# Autodesk Inventor assembly: GX 100
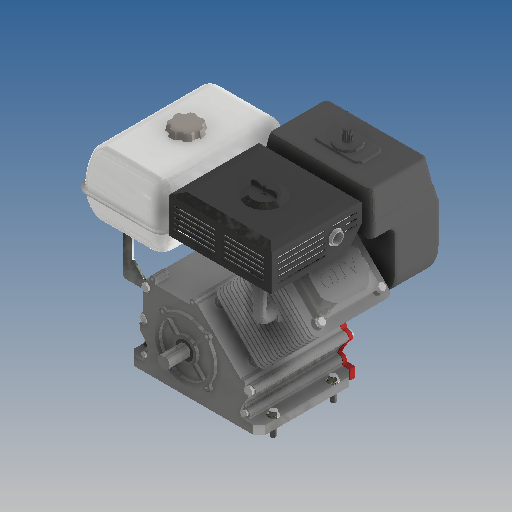
[picture p0: Inventor's stored thumbnail of the model, 512x512]
Saved by Autodesk Inventor 2021.1 (Build 251245000, 245)
## iProperties
Created: 2020-09-03
Part Number: GX 100
Document SubType Name: Assembly
Designer: alid
Description: Honda GX100 Engine
Author: alid
Revision Number: A
## Documents named in this file (3)
- C:\Vault Workspace\Design Data\Projects\PRJ0095\PWTR-CTO\PWTR-Supplier\GX 100.iam
- C:\Vault Workspace\Design Data\Projects\PRJ0095\PWTR-CTO\PWTR-Supplier\PWTR-0100.ipt
- C:\Vault Workspace\Design Data\Projects\PRJ0095\PWTR-CTO\PWTR-Supplier\PWTR-0134.ipt
## Components (5 placed, 2 different names)
1. EngineBlock — Insert:1
2. PWTR-0134:1 — Insert:1
3. PWTR-0134:2
4. PWTR-0134:3
5. PWTR-0134:4
## Component patterns: (4 elements, first: PWTR-0134:1)
## Relationships (1: Insert 1)
- Insert:1: EngineBlock ↔ PWTR-0134:1
